# Autodesk Inventor assembly: Vergaser_ra8846s
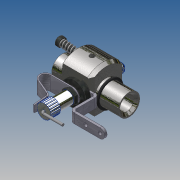
[picture p0: Inventor's stored thumbnail of the model, 180x180]
Saved by Autodesk Inventor 2021 (Build 250183000, 183)
## iProperties
Created: 2021-01-14
Part Number: Vergaser_ra8846s
Document SubType Name: Assembly
Designer: Sander
Author: Sander
## Documents named in this file (13)
- C:\Users\ricar\OneDrive - Fachhochschule Aachen\Mechatronik I\CAD\INVENTOR\Proyectos\Daten\Vergaser_ra8846s.iam
- C:\Users\ricar\OneDrive - Fachhochschule Aachen\Mechatronik I\CAD\INVENTOR\Proyectos\Daten\Vergasergehäuse_ra8846s.ipt
- C:\Users\ricar\OneDrive - Fachhochschule Aachen\Mechatronik I\CAD\INVENTOR\Proyectos\Daten\Einspritzdüse_ra8846s.ipt
- C:\Users\ricar\OneDrive - Fachhochschule Aachen\Mechatronik I\CAD\INVENTOR\Proyectos\Daten\Schließbahn_ra8846s.ipt
- C:\Users\ricar\OneDrive - Fachhochschule Aachen\Mechatronik I\CAD\INVENTOR\Proyectos\Daten\Gashebel_ra8846s.ipt
- C:\Users\ricar\OneDrive - Fachhochschule Aachen\Mechatronik I\CAD\INVENTOR\Proyectos\Daten\Dichtrign_ra8846s.ipt
- C:\Users\ricar\OneDrive - Fachhochschule Aachen\Mechatronik I\CAD\INVENTOR\Proyectos\Daten\Deckel_ra8846s.ipt
- C:\Users\ricar\OneDrive - Fachhochschule Aachen\Mechatronik I\CAD\INVENTOR\Proyectos\Daten\Rastfeder_ra8846s.ipt
- C:\Users\ricar\OneDrive - Fachhochschule Aachen\Mechatronik I\CAD\INVENTOR\Proyectos\Daten\Mutter_ra8846s.ipt
- C:\Users\ricar\OneDrive - Fachhochschule Aachen\Mechatronik I\CAD\INVENTOR\Proyectos\Daten\Nadelhalter_ra8846s.ipt
- C:\Users\ricar\OneDrive - Fachhochschule Aachen\Mechatronik I\CAD\INVENTOR\Proyectos\Daten\Düsennadel_ra8846s.ipt
- C:\Users\ricar\OneDrive - Fachhochschule Aachen\Mechatronik I\CAD\INVENTOR\Proyectos\Daten\Federundschraube_ra8846s.iam
- C:\Users\ricar\OneDrive - Fachhochschule Aachen\Mechatronik I\CAD\INVENTOR\Proyectos\Daten\O-Ring_ra8846s.ipt
## Components (13 placed, 12 different names)
1. Vergasergehäuse_ra8846s:1 — Winkel:1, Winkel:2, Winkel:3, Passend:5, Passend:6, Tangential:1, Tangential:2, Passend:7, Passend:8, Passend:9
2. Einspritzdüse_ra8846s:1 — Einfügen:1, Passend:8, Passend:9
3. Schließbahn_ra8846s:1 — Einfügen:1, Passend:2
4. Gashebel_ra8846s:1 — Passend:2, Einfügen:2, Winkel:1
5. Dichtrign_ra8846s:1 — Einfügen:2, Einfügen:3
6. Deckel_ra8846s:1 — Einfügen:3, Einfügen:4
7. Rastfeder_ra8846s:1 — Einfügen:4, Winkel:2, Einfügen:5
8. Mutter_ra8846s:1 — Einfügen:5, Einfügen:6
9. Nadelhalter_ra8846s:1 — Einfügen:6, Passend:3
10. Düsennadel_ra8846s:1 — Passend:3, Winkel:3
11. Federundschraube_ra8846s:1 [sub-assembly] — Passend:5, Tangential:2
12. Federundschraube_ra8846s:2 [sub-assembly] — Passend:6, Tangential:1
13. O-Ring_ra8846s:1 — Passend:7
## Relationships (18: Mate 7, Insert 6, Angle 3, Tangent 2)
- Einfügen:1 [Insert]: Einspritzdüse_ra8846s:1 ↔ Schließbahn_ra8846s:1
- Passend:2 [Mate]: Schließbahn_ra8846s:1 ↔ Gashebel_ra8846s:1
- Einfügen:2 [Insert]: Gashebel_ra8846s:1 ↔ Dichtrign_ra8846s:1
- Einfügen:3 [Insert]: Dichtrign_ra8846s:1 ↔ Deckel_ra8846s:1
- Winkel:1 [Angle] (0 deg): Vergasergehäuse_ra8846s:1 ↔ Gashebel_ra8846s:1
- Einfügen:4 [Insert]: Deckel_ra8846s:1 ↔ Rastfeder_ra8846s:1
- Winkel:2 [Angle] (0 deg): Vergasergehäuse_ra8846s:1 ↔ Rastfeder_ra8846s:1
- Einfügen:5 [Insert]: Rastfeder_ra8846s:1 ↔ Mutter_ra8846s:1
- Einfügen:6 [Insert]: Mutter_ra8846s:1 ↔ Nadelhalter_ra8846s:1
- Passend:3 [Mate]: Nadelhalter_ra8846s:1 ↔ Düsennadel_ra8846s:1
- Winkel:3 [Angle] (-90 deg): Vergasergehäuse_ra8846s:1 ↔ Düsennadel_ra8846s:1
- Passend:5 [Mate]: Vergasergehäuse_ra8846s:1 ↔ Federundschraube_ra8846s:1
- Passend:6 [Mate]: Vergasergehäuse_ra8846s:1 ↔ Federundschraube_ra8846s:2
- Tangential:1: Vergasergehäuse_ra8846s:1 ↔ Federundschraube_ra8846s:2
- Tangential:2: Vergasergehäuse_ra8846s:1 ↔ Federundschraube_ra8846s:1
- Passend:7 [Mate]: Vergasergehäuse_ra8846s:1 ↔ O-Ring_ra8846s:1
- Passend:8 [Mate]: Vergasergehäuse_ra8846s:1 ↔ Einspritzdüse_ra8846s:1
- Passend:9 [Mate]: Vergasergehäuse_ra8846s:1 ↔ Einspritzdüse_ra8846s:1
